# Autodesk Inventor assembly: Structure
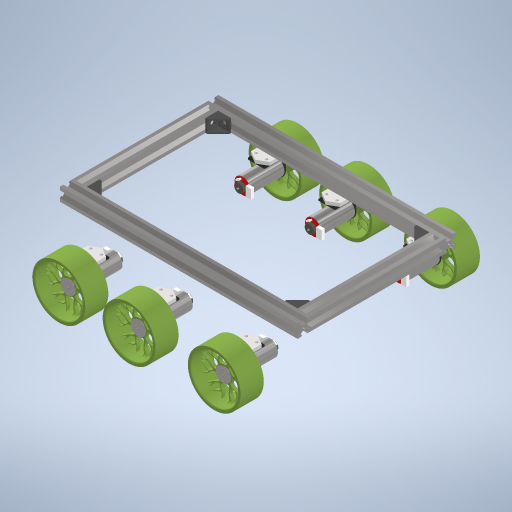
[picture p0: Inventor's stored thumbnail of the model, 512x512]
Saved by Autodesk Inventor 2024.2 (Build 282272000, 272)
## iProperties
Created: 2025-06-14
Part Number: Structure
Document SubType Name: Assembly
Designer: Admin
Author: Admin
## Documents named in this file (5)
- C:\Users\Admin\Documents\GitHub\ExplorateurErrant\Assemblies\main.iam
- C:\Users\Admin\Documents\GitHub\ExplorateurErrant\Structure\AluminumProfiles\ST-AluminumProfile-200.ipt
- C:\Users\Admin\Documents\GitHub\ExplorateurErrant\Structure\AluminumProfiles\ST-AluminumProfile-360.ipt
- C:\Users\Admin\Documents\GitHub\ExplorateurErrant\Structure\AluminumProfiles\ST-CornerBracket-2020.ipt
- C:\Users\Admin\Documents\GitHub\ExplorateurErrant\Assemblies\Wheel.iam
## Components (14 placed, 4 different names)
1. Wheel:1 [sub-assembly]
2. Wheel:2 [sub-assembly]
3. Wheel:3 [sub-assembly]
4. Wheel:4 [sub-assembly]
5. Wheel:5 [sub-assembly]
6. Wheel:6 [sub-assembly]
7. ST-AluminumProfile-200:1 — Mate:1, Flush:1, Flush:2, Mate:2, Mate:4, Flush:4, Flush:5, Mate:6
8. ST-AluminumProfile-360:1 — Mate:4, Flush:4, Flush:5, Mate:5, Flush:6, Mate:7, Flush:7, Flush:8, Mate:10, Flush:10
9. ST-AluminumProfile-360:2 — Mate:1, Flush:1, Flush:2, Mate:3, Flush:3, Mate:8, Flush:9
10. ST-CornerBracket-2020:1 — Mate:10, Mate:11, Flush:10
11. ST-CornerBracket-2020:2 — Mate:5, Mate:6, Flush:6
12. ST-CornerBracket-2020:3 — Mate:2, Mate:3, Flush:3
13. ST-CornerBracket-2020:4 — Mate:8, Mate:9, Flush:9
14. ST-AluminumProfile-200:2 — Mate:7, Flush:7, Flush:8, Mate:9, Mate:11
## Relationships (21: Mate 11, Flush 10)
- Mate:1: ST-AluminumProfile-200:1 ↔ ST-AluminumProfile-360:2
- Flush:1: ST-AluminumProfile-200:1 ↔ ST-AluminumProfile-360:2
- Flush:2: ST-AluminumProfile-200:1 ↔ ST-AluminumProfile-360:2
- Mate:2: ST-AluminumProfile-200:1 ↔ ST-CornerBracket-2020:3
- Mate:3: ST-AluminumProfile-360:2 ↔ ST-CornerBracket-2020:3
- Flush:3: ST-AluminumProfile-360:2 ↔ ST-CornerBracket-2020:3
- Mate:4: ST-AluminumProfile-200:1 ↔ ST-AluminumProfile-360:1
- Flush:4: ST-AluminumProfile-200:1 ↔ ST-AluminumProfile-360:1
- Flush:5: ST-AluminumProfile-200:1 ↔ ST-AluminumProfile-360:1
- Mate:5: ST-AluminumProfile-360:1 ↔ ST-CornerBracket-2020:2
- Mate:6: ST-AluminumProfile-200:1 ↔ ST-CornerBracket-2020:2
- Flush:6: ST-AluminumProfile-360:1 ↔ ST-CornerBracket-2020:2
- Mate:7: ST-AluminumProfile-360:1 ↔ ST-AluminumProfile-200:2
- Flush:7: ST-AluminumProfile-360:1 ↔ ST-AluminumProfile-200:2
- Flush:8: ST-AluminumProfile-360:1 ↔ ST-AluminumProfile-200:2
- Mate:8: ST-AluminumProfile-360:2 ↔ ST-CornerBracket-2020:4
- Mate:9: ST-CornerBracket-2020:4 ↔ ST-AluminumProfile-200:2
- Flush:9: ST-AluminumProfile-360:2 ↔ ST-CornerBracket-2020:4
- Mate:10: ST-AluminumProfile-360:1 ↔ ST-CornerBracket-2020:1
- Mate:11: ST-CornerBracket-2020:1 ↔ ST-AluminumProfile-200:2
- Flush:10: ST-AluminumProfile-360:1 ↔ ST-CornerBracket-2020:1
